# Autodesk Inventor assembly: UNLHEP-14-A-01-002_GantryChuckWplate
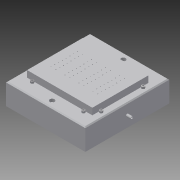
[picture p0: Inventor's stored thumbnail of the model, 180x180]
Saved by Autodesk Inventor 2013 (Build 170138000, 138)
## iProperties
Created: 2014-01-13
Part Number: UNLHEP-14-A-01-002_GantryChuckWplate
Document SubType Name: Assembly
Designer: Frank Meier
Project: UNL Pixel Phase I
Author: Frank Meier
## Documents named in this file (6)
- C:\Users\Frank Meier\Documents\Inventor\Delvotec-Saugplatte\UNLHEP-14-01-A-002_GantryChuckWplate.iam
- C:\Users\Frank Meier\Documents\Inventor\Delvotec-Saugplatte\UNLHEP-14-01-P-004_ChuckForGantry.ipt
- C:\Users\Frank Meier\Documents\Inventor\Delvotec-Saugplatte\UNLHEP-14-01-P-001_ModuleChuck.ipt
- C:\Users\Frank Meier\Documents\Inventor\Content Center Files\R2013\de-DE\ISO 4762(2)\ISO 4762 - M4 x 10ISO.ipt
- C:\Users\Frank Meier\Documents\Inventor\Content Center Files\R2013\de-DE\ISO 4762(2)\ISO 4762 - M4 x 6ISO.ipt
- C:\Users\Frank Meier\Documents\Inventor\Delvotec-Saugplatte\UNLHEP-14-01-P-003_Tube4mmID20mm.ipt
## Components (11 placed, 5 different names)
1. UNLHEP-14-01-P-001_ChuckForGantry:1 — Passend:1, Einfügen:8, Einfügen:9, Einfügen:10, Einfügen:11, Einfügen:12, Einfügen:13, Einfügen:14, Einfügen:15, Passend:5, Passend:6
2. UNLHEP-14-01-P-001_ModuleChuck:1 — Passend:1, Passend:2, Passend:3, Passend:4
3. ISO 4762 M4 x 10:1 — Einfügen:8
4. ISO 4762 M4 x 6:1 — Einfügen:9, Passend:4
5. ISO 4762 M4 x 6:2 — Einfügen:10, Passend:2
6. ISO 4762 M4 x 6:3 — Einfügen:11, Passend:3
7. ISO 4762 M4 x 6:4 — Einfügen:12
8. ISO 4762 M4 x 6:5 — Einfügen:13
9. ISO 4762 M4 x 6:6 — Einfügen:14
10. ISO 4762 M4 x 6:7 — Einfügen:15
11. UNLHEP-14-01-P-003_Tube4mmID20mm:1 — Passend:5, Passend:6
## Relationships (14: Insert 8, Mate 6)
- Passend:1 [Mate]: UNLHEP-14-01-P-001_ChuckForGantry:1 ↔ UNLHEP-14-01-P-001_ModuleChuck:1
- Passend:2 [Mate] (3.5 mm): UNLHEP-14-01-P-001_ModuleChuck:1 ↔ ISO 4762 M4 x 6:2
- Passend:3 [Mate] (3.5 mm): UNLHEP-14-01-P-001_ModuleChuck:1 ↔ ISO 4762 M4 x 6:3
- Passend:4 [Mate] (3.5 mm): UNLHEP-14-01-P-001_ModuleChuck:1 ↔ ISO 4762 M4 x 6:1
- Passend:5 [Mate]: UNLHEP-14-01-P-001_ChuckForGantry:1 ↔ UNLHEP-14-01-P-003_Tube4mmID20mm:1
- Passend:6 [Mate]: UNLHEP-14-01-P-001_ChuckForGantry:1 ↔ UNLHEP-14-01-P-003_Tube4mmID20mm:1
- Einfügen:8 [Insert]: UNLHEP-14-01-P-001_ChuckForGantry:1 ↔ ISO 4762 M4 x 10:1
- Einfügen:9 [Insert]: UNLHEP-14-01-P-001_ChuckForGantry:1 ↔ ISO 4762 M4 x 6:1
- Einfügen:10 [Insert]: UNLHEP-14-01-P-001_ChuckForGantry:1 ↔ ISO 4762 M4 x 6:2
- Einfügen:11 [Insert]: UNLHEP-14-01-P-001_ChuckForGantry:1 ↔ ISO 4762 M4 x 6:3
- Einfügen:12 [Insert]: UNLHEP-14-01-P-001_ChuckForGantry:1 ↔ ISO 4762 M4 x 6:4
- Einfügen:13 [Insert]: UNLHEP-14-01-P-001_ChuckForGantry:1 ↔ ISO 4762 M4 x 6:5
- Einfügen:14 [Insert]: UNLHEP-14-01-P-001_ChuckForGantry:1 ↔ ISO 4762 M4 x 6:6
- Einfügen:15 [Insert]: UNLHEP-14-01-P-001_ChuckForGantry:1 ↔ ISO 4762 M4 x 6:7
